# Autodesk Inventor assembly: VEXpro-VersaPlanetary-2stage-with-BAG
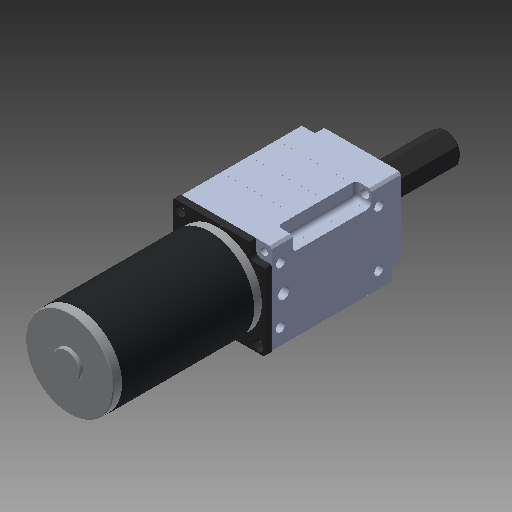
[picture p0: Inventor's stored thumbnail of the model, 512x512]
Saved by Autodesk Inventor 2017 (Build 210142000, 142)
## iProperties
Created: 2014-02-17
Part Number: VEXpro-VersaPlanetary-2stage-with-BAG
Description: STEP AP214
Document SubType Name: Assembly
Designer: Hanson
Sending System: SolidWorks 2013
Preprocessor: SwSTEP 2.0
Title: BAG 2 stage Release.STEP
Author: IFMI-VEX04
Revision Number: ANY
## Documents named in this file (21)
- \\Mac\Home\Desktop\bunnybots 2016\15102898-16-Bunnybot-CAD\Bunnybot-To_be_renamed\15102898-16-A-0000\15102898-16-A-0600\VEXpro-VersaPlanetary-2stage-with-BAG.iam
- \\Mac\Home\Desktop\bunnybots 2016\15102898-16-Bunnybot-CAD\Bunnybot-To_be_renamed\15102898-16-A-0000\15102898-16-A-0300\Imported Components\BAG motor\217-2625-001 Rev1.ipt
- \\Mac\Home\Desktop\bunnybots 2016\15102898-16-Bunnybot-CAD\Bunnybot-To_be_renamed\15102898-16-A-0000\15102898-16-A-0300\Imported Components\BAG motor\217-2625-002 Rev1.ipt
- \\Mac\Home\Desktop\bunnybots 2016\15102898-16-Bunnybot-CAD\Bunnybot-To_be_renamed\15102898-16-A-0000\15102898-16-A-0300\Imported Components\BAG motor\217-2625-003 Rev1.ipt
- \\Mac\Home\Desktop\bunnybots 2016\15102898-16-Bunnybot-CAD\Bunnybot-To_be_renamed\15102898-16-A-0000\15102898-16-A-0300\Imported Components\BAG motor\217-2625-009 Rev1.ipt
- E:\CAD\Bag motor\217-2625-100.iam
- E:\CAD\Bag motor\217-2625-007 Rev1_Sun_Driver01.ipt
- E:\CAD\Bag motor\217-2742.ipt
- E:\CAD\Bag motor\217-2741.ipt
- E:\CAD\Bag motor\TRUARC-MSH-15_98541A410.ipt
- E:\CAD\Bag motor\SPRGW0856-1102-012_9714K62.ipt
- \\Mac\Home\Desktop\bunnybots 2016\15102898-16-Bunnybot-CAD\Bunnybot-To_be_renamed\15102898-16-A-0000\15102898-16-A-0300\Imported Components\BAG motor\SSS1032-0125ZB_94105A824.ipt
- E:\CAD\Bag motor\TRUARC-5103-68_97414A675_grv.ipt
- \\Mac\Home\Desktop\bunnybots 2016\15102898-16-Bunnybot-CAD\Bunnybot-To_be_renamed\15102898-16-A-0000\15102898-16-A-0300\Imported Components\BAG motor\217-3351.ipt
- \\Mac\Home\Desktop\bunnybots 2016\15102898-16-Bunnybot-CAD\Bunnybot-To_be_renamed\15102898-16-A-0000\15102898-16-A-0300\Imported Components\BAG motor\217-2816-001 Rev1.ipt
- E:\CAD\Bag motor\SSA_SSA0832-1750ZC.ipt
- \\Mac\Home\Desktop\bunnybots 2016\15102898-16-Bunnybot-CAD\Bunnybot-To_be_renamed\15102898-16-A-0000\15102898-16-A-0300\Imported Components\BAG motor\217-2625-011 Rev1.ipt
- E:\CAD\Bag motor\SSA_SSA0832-0500ZC.ipt
- E:\CAD\Bag motor\SSHCM004_SSHCM004070010C.ipt
- E:\CAD\Bag motor\217-2818 Rev1.iam
- \\Mac\Home\Desktop\bunnybots 2016\15102898-16-Bunnybot-CAD\Bunnybot-To_be_renamed\15102898-16-A-0000\15102898-16-A-0300\Imported Components\BAG motor\217-2822-003 Rev4.ipt
## Components (25 placed, 25 different names)
1. 217-2625-001 Rev1_1
2. 217-2625-002 Rev1_2
3. 217-2625-003 Rev1_3 — Insert:1
4. 217-2625-009 Rev1_4
5. 217-2625-100_5 [sub-assembly]
6. 217-2625-007 Rev1_Sun_Driver01_6
7. 217-2742_7 — Insert:1
8. 217-2742_8
9. 217-2741_9
10. TRUARC-MSH-15_98541A410_10
11. SPRGW0856-1102-012_9714K62_11
12. SSS1032-0125ZB_94105A824_12
13. TRUARC-5103-68_97414A675_grv_13
14. 217-3351_14
15. 217-2816-001 Rev1_15
16. SSA_SSA0832-1750ZC_16
17. SSA_SSA0832-1750ZC_17
18. 217-2625-011 Rev1_18
19. SSA_SSA0832-0500ZC_19
20. SSA_SSA0832-0500ZC_20
21. SSHCM004_SSHCM004070010C_21
22. SSHCM004_SSHCM004070010C_22
23. 217-2816-001 Rev1_23
24. 217-2818 Rev1_24 [sub-assembly]
25. 217-2822-003 Rev4_25
## Relationships (1: Insert 1)
- Insert:1: 217-2625-003 Rev1_3 ↔ 217-2742_7
